# Autodesk Inventor assembly: Claw_1
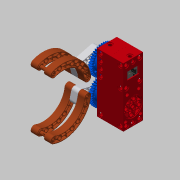
[picture p0: Inventor's stored thumbnail of the model, 180x180]
Saved by Autodesk Inventor 2019.3 (Build 233278000, 278)
## iProperties
Created: 2019-03-18
Part Number: Claw_1
Document SubType Name: Assembly
Designer: Varga Daniel
Author: Varga Daniel
## Documents named in this file (8)
- C:\!_Dani\!_cloud\OneDrive\!_munka\Revolution\RevvyDemoKit\Structural parts\Test assemblies\Claw_big_3_double.iam
- C:\!_Dani\!_cloud\OneDrive\!_munka\Revolution\RevvyDemoKit\Structural parts\Connetor Pins\CP1+x1+\CP1x1.ipt
- C:\!_Dani\!_cloud\OneDrive\!_munka\Revolution\RevvyDemoKit\Structural parts\Gears\G40.ipt
- C:\!_Dani\!_cloud\OneDrive\!_munka\Revolution\RevvyDemoKit\Structural parts\Demo parts\Motor\Inventor imported\motor.iam
- C:\!_Dani\!_cloud\OneDrive\!_munka\Revolution\RevvyDemoKit\Structural parts\Axles\AXp2p.ipt
- C:\!_Dani\!_cloud\OneDrive\!_munka\Revolution\RevvyDemoKit\Structural parts\Beams\Straight Beams\S2+x2\S4x2.ipt
- C:\!_Dani\!_cloud\OneDrive\!_munka\Revolution\RevvyDemoKit\Structural parts\Connetor Pins\CP1+x1+\CP2x1.ipt
- C:\!_Dani\!_cloud\OneDrive\!_munka\Revolution\RevvyDemoKit\Structural parts\Beams\Curved beams\CB6H.ipt
## Components (21 placed, 7 different names)
1. G40:1 — Mate:6, Angle:1, Rotation:1, Insert:34, Insert:35, Insert:36
2. motor:1 [sub-assembly] — Mate:1, Flush:1, Mate:2, Mate:6, Angle:2, Mate:10, Insert:43
3. CB6H:2 — Insert:30, Mate:9
4. AXp2p:1 — Mate:3, Mate:4, Insert:43, Mate:11
5. G40:2 — Mate:3, Mate:4, Angle:1, Angle:2, Rotation:1, Insert:39, Insert:40, Mate:11
6. CB6H:1 — Insert:29, Mate:8
7. S4x2:1 — Insert:37, Insert:38
8. S4x2:2 — Insert:41, Insert:42
9. CP2x1:3
10. CP2x1:2
11. CP2x1:4
12. CP2x1:5
13. CB6H:3 — Insert:32, Mate:8
14. CB6H:4 — Insert:33, Mate:9
15. CP2x1:6 — Insert:29, Insert:32
16. CP2x1:7 — Insert:30, Insert:33
17. CP2x1:8 — Insert:36, Insert:37
18. CP1x1:11 — Insert:35, Insert:38
19. CP1x1:12 — Insert:34, Mate:10
20. CP1x1:13 — Insert:40, Insert:41
21. CP1x1:14 — Insert:39, Insert:42
## Relationships (35: Insert 22, Mate 9, Angle 2, Flush 1, RelateRotation 1)
- Mate:1: motor:1
- Flush:1: motor:1
- Mate:2: motor:1
- Mate:3: AXp2p:1 ↔ G40:2
- Mate:4: AXp2p:1 ↔ G40:2
- Mate:6: G40:1 ↔ motor:1
- Angle:1 (0 deg): G40:1 ↔ G40:2
- Angle:2 (0 deg): motor:1 ↔ G40:2
- [Insert]: S4x2:1 ↔ CP2x1:3
- [Insert]: S4x2:1 ↔ CP2x1:2
- [Insert]: CB6H:1 ↔ CP2x1:3
- [Insert]: CB6H:1 ↔ CP2x1:2
- [Insert]: S4x2:2 ↔ CP2x1:4
- [Insert]: S4x2:2 ↔ CP2x1:5
- [Insert]: CB6H:2 ↔ CP2x1:4
- [Insert]: CB6H:2 ↔ CP2x1:5
- Rotation:1 [RelateRotation] (1 ul): G40:1 ↔ G40:2
- Insert:29: CB6H:1 ↔ CP2x1:6
- Insert:30: CB6H:2 ↔ CP2x1:7
- Insert:32: CB6H:3 ↔ CP2x1:6
- Mate:8: CB6H:1 ↔ CB6H:3
- Insert:33: CB6H:4 ↔ CP2x1:7
- Mate:9: CB6H:2 ↔ CB6H:4
- Insert:34: G40:1 ↔ CP1x1:12
- Insert:35: G40:1 ↔ CP1x1:11
- Insert:36: G40:1 ↔ CP2x1:8
- Insert:37: S4x2:1 ↔ CP2x1:8
- Insert:38: S4x2:1 ↔ CP1x1:11
- Insert:39: G40:2 ↔ CP1x1:14
- Insert:40: G40:2 ↔ CP1x1:13
- Insert:41: S4x2:2 ↔ CP1x1:13
- Insert:42: S4x2:2 ↔ CP1x1:14
- Mate:10: motor:1 ↔ CP1x1:12
- Insert:43: motor:1 ↔ AXp2p:1
- Mate:11: AXp2p:1 ↔ G40:2
